# Autodesk Inventor assembly: x2010-8-FIRSTwheel-END
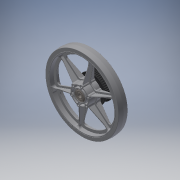
[picture p0: Inventor's stored thumbnail of the model, 180x180]
Saved by Autodesk Inventor 2016 (Build 200138000, 138)
## iProperties
Company: Unknown
Created: 2016-01-13
Part Number: x2010-8-FIRSTwheel-END
Description: Unknown
Document SubType Name: Assembly
Designer: Douglas
Sending System: Unknown
Preprocessor: XStep 1.0
Title: //Amserv/amserver/AndyMark/Products/Wheels Solid/FIRST Wheel 2010 8 inch/2010 8 wheel.stp
Author: Unknown
Revision Number: NONE
## Documents named in this file (6)
- D:\SkyDrive\GitHub\2016-Robot-CAD\Inventor\PARTS\x2010-8-FIRSTwheel-END.iam
- D:\SkyDrive\GitHub\2016-Robot-CAD\Inventor\PARTS\2010 8 tread.ipt
- D:\SkyDrive\GitHub\2016-Robot-CAD\Inventor\PARTS\2010 8 hub.ipt
- D:\SkyDrive\GitHub\2016-Robot-CAD\Inventor\Chassis\42 tooth HTD Pulley half 2014.ipt
- D:\SkyDrive\GitHub\2016-Robot-CAD\Inventor\Chassis\10-24 Hex Washer Rolling x 1.25_93882A213.ipt
- D:\SkyDrive\GitHub\2016-Robot-CAD\Inventor\Chassis\1614Z Bearing.ipt
## Components (12 placed, 5 different names)
1. 2010 8 tread — Mate:4, Flush:1
2. 2010 8 hub — Mate:4, Flush:1, Mate:11, Mate:12, Mate:13, Mate:33, Mate:34
3. 42 tooth HTD Pulley half 2014:3 — Mate:19, Mate:20, Mate:21, Mate:22, Mate:23, Mate:24, Mate:25, Mate:26, Mate:27, Mate:28, Mate:29, Mate:30, Mate:31, Mate:32
4. 42 tooth HTD Pulley half 2014:4 — Mate:11, Mate:12, Mate:13
5. 10-24 Hex Washer Rolling x 1.25_93882A213:1 — Mate:19, Mate:20
6. 10-24 Hex Washer Rolling x 1.25_93882A213:2 — Mate:21, Mate:22
7. 10-24 Hex Washer Rolling x 1.25_93882A213:3 — Mate:23, Mate:24
8. 10-24 Hex Washer Rolling x 1.25_93882A213:4 — Mate:29, Mate:30
9. 10-24 Hex Washer Rolling x 1.25_93882A213:8 — Mate:25, Mate:26
10. 10-24 Hex Washer Rolling x 1.25_93882A213:12 — Mate:27, Mate:28
11. 1614Z Bearing:1 — Mate:31, Mate:32
12. 1614Z Bearing:2 — Mate:33, Mate:34
## Relationships (24: Mate 23, Flush 1)
- Mate:4: 2010 8 tread ↔ 2010 8 hub
- Flush:1: 2010 8 tread ↔ 2010 8 hub
- [Mate]: 42 tooth HTD Pulley half 2014:3 ↔ 42 tooth HTD Pulley half 2014:4
- [Mate]: 42 tooth HTD Pulley half 2014:3 ↔ 42 tooth HTD Pulley half 2014:4
- [Mate]: 42 tooth HTD Pulley half 2014:3 ↔ 42 tooth HTD Pulley half 2014:4
- Mate:11: 2010 8 hub ↔ 42 tooth HTD Pulley half 2014:4
- Mate:12: 2010 8 hub ↔ 42 tooth HTD Pulley half 2014:4
- Mate:13: 2010 8 hub ↔ 42 tooth HTD Pulley half 2014:4
- Mate:19: 42 tooth HTD Pulley half 2014:3 ↔ 10-24 Hex Washer Rolling x 1.25_93882A213:1
- Mate:20: 42 tooth HTD Pulley half 2014:3 ↔ 10-24 Hex Washer Rolling x 1.25_93882A213:1
- Mate:21: 42 tooth HTD Pulley half 2014:3 ↔ 10-24 Hex Washer Rolling x 1.25_93882A213:2
- Mate:22: 42 tooth HTD Pulley half 2014:3 ↔ 10-24 Hex Washer Rolling x 1.25_93882A213:2
- Mate:23: 42 tooth HTD Pulley half 2014:3 ↔ 10-24 Hex Washer Rolling x 1.25_93882A213:3
- Mate:24: 42 tooth HTD Pulley half 2014:3 ↔ 10-24 Hex Washer Rolling x 1.25_93882A213:3
- Mate:25: 42 tooth HTD Pulley half 2014:3 ↔ 10-24 Hex Washer Rolling x 1.25_93882A213:8
- Mate:26: 42 tooth HTD Pulley half 2014:3 ↔ 10-24 Hex Washer Rolling x 1.25_93882A213:8
- Mate:27: 42 tooth HTD Pulley half 2014:3 ↔ 10-24 Hex Washer Rolling x 1.25_93882A213:12
- Mate:28: 42 tooth HTD Pulley half 2014:3 ↔ 10-24 Hex Washer Rolling x 1.25_93882A213:12
- Mate:29: 42 tooth HTD Pulley half 2014:3 ↔ 10-24 Hex Washer Rolling x 1.25_93882A213:4
- Mate:30: 42 tooth HTD Pulley half 2014:3 ↔ 10-24 Hex Washer Rolling x 1.25_93882A213:4
- Mate:31: 42 tooth HTD Pulley half 2014:3 ↔ 1614Z Bearing:1
- Mate:32: 42 tooth HTD Pulley half 2014:3 ↔ 1614Z Bearing:1
- Mate:33: 2010 8 hub ↔ 1614Z Bearing:2
- Mate:34: 2010 8 hub ↔ 1614Z Bearing:2
## Named parameters: d8_d0 = 0 mm, d9_d1 = 0 mm, d10_d2 = 0 mm
